# Autodesk Inventor assembly: Пандус
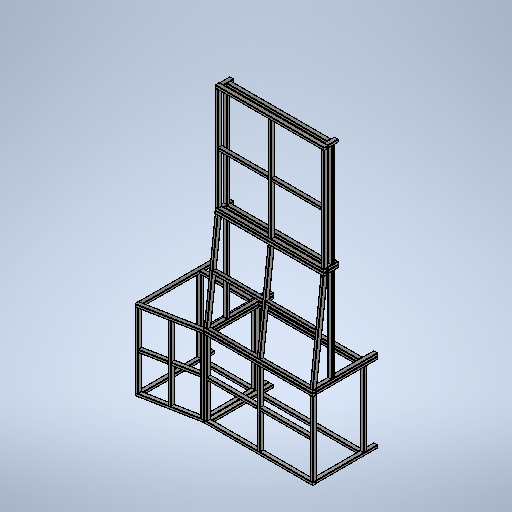
[picture p0: Inventor's stored thumbnail of the model, 512x512]
Saved by Autodesk Inventor 2025 (Build 290162010, 162A)
## iProperties
Created: 2024-09-18
Part Number: Пандус
Document SubType Name: Assembly
Designer: pokla
Author: pokla
## Documents named in this file (13)
- C:\Users\pokla\Documents\Inventor\BSH_Beshkino_bio_tank\Пандус.iam
- C:\Users\pokla\Documents\Inventor\BSH_Beshkino_bio_tank\Тумба 2.iam
- C:\Users\pokla\Documents\Inventor\BSH_Beshkino_bio_tank\Ноги тумба 2.iam
- C:\Users\pokla\Documents\Inventor\BSH_Beshkino_bio_tank\Тумба 4.iam
- C:\Users\pokla\Documents\Inventor\BSH_Beshkino_bio_tank\Ноги тумба 4.iam
- C:\Users\pokla\Documents\Inventor\BSH_Beshkino_bio_tank\Тумба 3.iam
- C:\Users\pokla\Documents\Inventor\BSH_Beshkino_bio_tank\Нога тумба 3.1.iam
- C:\Users\pokla\Documents\Inventor\BSH_Beshkino_bio_tank\Нога тумба 3.2.iam
- C:\Users\pokla\Documents\Inventor\BSH_Beshkino_bio_tank\Тумба 1.iam
- C:\Users\pokla\Documents\Inventor\BSH_Beshkino_bio_tank\Ноги тумба 1.iam
- C:\Users\pokla\Documents\Inventor\BSH_Beshkino_bio_tank\ISO 4019 - 60x40x3 - 691.ipt
- C:\Users\pokla\Documents\Inventor\BSH_Beshkino_bio_tank\ISO 4019 - 60x40x3 - 1380.ipt
- C:\Users\pokla\Documents\Inventor\BSH_Beshkino_bio_tank\ISO 4019 - 60x40x3 - 1286,407.ipt
## Components (20 placed, 12 different names)
1. Тумба 2:1 [sub-assembly]
2. Ноги тумба 2:1 [sub-assembly]
3. Ноги тумба 2:2 [sub-assembly] — Mate:5, Flush:10, Flush:11, Mate:6, Flush:12, Flush:13
4. Тумба 4:1 [sub-assembly]
5. Ноги тумба 4:1 [sub-assembly] — Mate:7, Flush:14, Flush:15, Mate:8, Flush:16, Flush:17
6. Ноги тумба 4:2 [sub-assembly]
7. Тумба 3:1 [sub-assembly]
8. Нога тумба 3.1:1 [sub-assembly]
9. Нога тумба 3.2:1 [sub-assembly] — Mate:9, Flush:18, Flush:19, Mate:10, Flush:20, Flush:21
10. Тумба 1:1 [sub-assembly]
11. Ноги тумба 2:3 [sub-assembly]
12. Ноги тумба 1:1 [sub-assembly] — Mate:3, Flush:6, Flush:7, Mate:4, Flush:8, Flush:9
13. ISO 4019 - 60x40x3 - 691:1 — Mate:3, Flush:6, Flush:7
14. ISO 4019 - 60x40x3 - 691:2 — Mate:4, Flush:8, Flush:9
15. ISO 4019 - 60x40x3 - 1380:1 — Mate:5, Flush:10, Flush:11
16. ISO 4019 - 60x40x3 - 1380:2 — Mate:6, Flush:12, Flush:13
17. ISO 4019 - 60x40x3 - 1380:3 — Mate:7, Flush:14, Flush:15
18. ISO 4019 - 60x40x3 - 1380:4 — Mate:8, Flush:16, Flush:17
19. ISO 4019 - 60x40x3 - 1286,407:1 — Mate:9, Flush:18, Flush:19
20. ISO 4019 - 60x40x3 - 1286,407:2 — Mate:10, Flush:20, Flush:21
## Relationships (44: Flush 21, Mate 10, WeldJoint 7, Tangent 6)
- [WeldJoint]: Тумба 2:1 ↔ Ноги тумба 2:1
- [WeldJoint]: Тумба 2:1 ↔ Ноги тумба 2:2
- [WeldJoint]: Тумба 4:1 ↔ Ноги тумба 4:1
- [WeldJoint]: Тумба 4:1 ↔ Ноги тумба 4:2
- [WeldJoint]: Ноги тумба 2:1 ↔ Нога тумба 3.1:1
- [WeldJoint]: Ноги тумба 4:1 ↔ Нога тумба 3.2:1
- [Flush]: Тумба 2:1 ↔ Тумба 4:1
- [Tangent]: Тумба 3:1 ↔ Нога тумба 3.2:1
- [Tangent]: Тумба 3:1 ↔ Нога тумба 3.1:1
- [Flush]: Тумба 2:1 ↔ Тумба 3:1
- [Tangent]: Тумба 4:1 ↔ Тумба 3:1
- [Tangent]: Тумба 2:1 ↔ Тумба 3:1
- [WeldJoint]: Ноги тумба 2:2 ↔ Ноги тумба 2:3
- [Flush]: Ноги тумба 2:2 ↔ Ноги тумба 1:1
- [Flush]: Ноги тумба 2:3 ↔ Ноги тумба 1:1
- [Flush]: Тумба 1:1 ↔ Ноги тумба 2:3
- [Mate] (691 mm): Ноги тумба 2:3 ↔ Ноги тумба 1:1
- [Tangent]: Тумба 1:1 ↔ Ноги тумба 2:3
- [Tangent]: Тумба 1:1 ↔ Ноги тумба 1:1
- [Mate]: Тумба 1:1 ↔ Ноги тумба 1:1
- Mate:3: Ноги тумба 1:1 ↔ ISO 4019 - 60x40x3 - 691:1
- Flush:6 (150 mm): Ноги тумба 1:1 ↔ ISO 4019 - 60x40x3 - 691:1
- Flush:7: Ноги тумба 1:1 ↔ ISO 4019 - 60x40x3 - 691:1
- Mate:4: Ноги тумба 1:1 ↔ ISO 4019 - 60x40x3 - 691:2
- Flush:8: Ноги тумба 1:1 ↔ ISO 4019 - 60x40x3 - 691:2
- Flush:9 (150 mm): Ноги тумба 1:1 ↔ ISO 4019 - 60x40x3 - 691:2
- Mate:5: Ноги тумба 2:2 ↔ ISO 4019 - 60x40x3 - 1380:1
- Flush:10: Ноги тумба 2:2 ↔ ISO 4019 - 60x40x3 - 1380:1
- Flush:11 (150 mm): Ноги тумба 2:2 ↔ ISO 4019 - 60x40x3 - 1380:1
- Mate:6: Ноги тумба 2:2 ↔ ISO 4019 - 60x40x3 - 1380:2
- Flush:12: Ноги тумба 2:2 ↔ ISO 4019 - 60x40x3 - 1380:2
- Flush:13 (150 mm): Ноги тумба 2:2 ↔ ISO 4019 - 60x40x3 - 1380:2
- Mate:7: Ноги тумба 4:1 ↔ ISO 4019 - 60x40x3 - 1380:3
- Flush:14: Ноги тумба 4:1 ↔ ISO 4019 - 60x40x3 - 1380:3
- Flush:15 (40 mm): Ноги тумба 4:1 ↔ ISO 4019 - 60x40x3 - 1380:3
- Mate:8: Ноги тумба 4:1 ↔ ISO 4019 - 60x40x3 - 1380:4
- Flush:16: Ноги тумба 4:1 ↔ ISO 4019 - 60x40x3 - 1380:4
- Flush:17 (40 mm): Ноги тумба 4:1 ↔ ISO 4019 - 60x40x3 - 1380:4
- Mate:9: Нога тумба 3.2:1 ↔ ISO 4019 - 60x40x3 - 1286,407:1
- Flush:18: Нога тумба 3.2:1 ↔ ISO 4019 - 60x40x3 - 1286,407:1
- Flush:19 (50 mm): Нога тумба 3.2:1 ↔ ISO 4019 - 60x40x3 - 1286,407:1
- Mate:10: Нога тумба 3.2:1 ↔ ISO 4019 - 60x40x3 - 1286,407:2
- Flush:20: Нога тумба 3.2:1 ↔ ISO 4019 - 60x40x3 - 1286,407:2
- Flush:21 (50 mm): Нога тумба 3.2:1 ↔ ISO 4019 - 60x40x3 - 1286,407:2
